# Autodesk Inventor assembly: Ekran
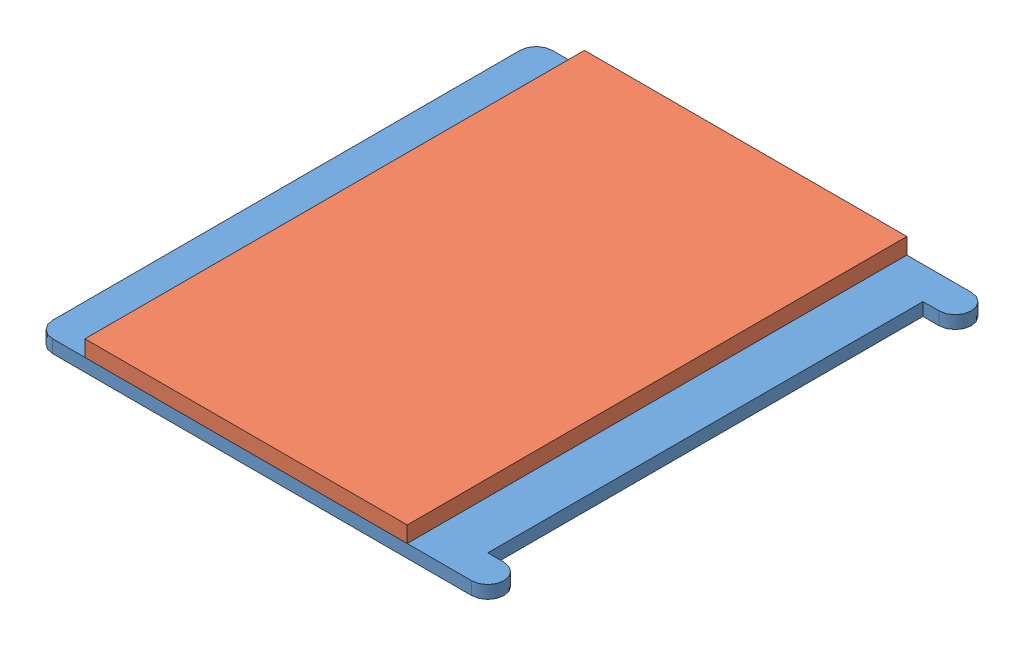
[picture p0: shaded view drawn from the part files that the assembly names]
Saved by Autodesk Inventor 2025 (Build 290162000, 162)
## iProperties
Created: 2024-04-15
Part Number: Ekran
Document SubType Name: Assembly
Designer: sicia
Author: sicia
## Documents named in this file (3)
- D:\Dokumenty\GitHub\ESP32_tracker\hardware\Ekran.iam
- D:\Dokumenty\GitHub\ESP32_tracker\hardware\Płytka.ipt
- D:\Dokumenty\GitHub\ESP32_tracker\hardware\Szkło.ipt
## Components (2 placed, 2 different names)
1. Płytka:1 — Flush:1, Flush:2
2. Szkło:1 — Flush:1, Flush:2
## Relationships (2: Flush 2)
- Flush:1: Płytka:1 ↔ Szkło:1
- Flush:2: Płytka:1 ↔ Szkło:1
